# Autodesk Inventor assembly: BeltDrive
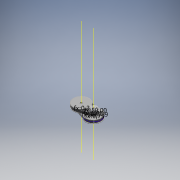
[picture p0: Inventor's stored thumbnail of the model, 180x180]
Saved by Autodesk Inventor 2018.3 (Build 223284000, 284)
## iProperties
Created: 2018-07-29
Part Number: BeltDrive
Material: Generisch
Document SubType Name: Assembly
Designer: JochenAlt
Author: JochenAlt
## Documents named in this file (10)
- D:\Projects\FlowerPot\CAD\Beltdrive\BeltDrive.iam
- D:\Projects\FlowerPot\CAD\Mounting Hub.ipt
- D:\Projects\FlowerPot\CAD\Beltdrive\ZwischenScheibe.ipt
- D:\Projects\FlowerPot\CAD\AST_Bearings_SMR74ZZ.ipt
- D:\Projects\FlowerPot\CAD\Beltdrive\BeltDriveConstruction\Konstruktions-Assistent\Synchrone Riemenscheibe22.ipt
- D:\Projects\FlowerPot\CAD\Beltdrive\Konstruktions-Assistent\Synchrone Riemenscheibe21.ipt
- D:\Projects\FlowerPot\CAD\Beltdrive\Konstruktions-Assistent\Zahnriemen1.ipt
- D:\Projects\FlowerPot\CAD\Beltdrive\BeltDriveConstruction\Konstruktions-Assistent\Zahnriemen2.ipt
- C:\Users\JochenAlt\Documents\Inventor\Content Center Files\R2018\de-DE\DIN 912\DIN 912 - M2,5 x 0,45 x 12 x 10,875.ipt
- C:\Users\JochenAlt\Documents\Inventor\Content Center Files\R2018\de-DE\DIN 912\DIN 912 - M3 x 0,5 x 6 x 4,75.ipt
## Components (17 placed, 8 different names)
1. Mounting Hub:1 — Passend:17, Passend:18, Passend:19, Passend:30
2. BigWheel — Passend:26, Passend:27, Passend:29, Drehung:1, Drehung:2, Fluchtend:2, Fluchtend:3
3. Mounting Hub:2 — Passend:5, Passend:6, Passend:21, Passend:32
4. AST_Bearings_SMR74ZZ:2 — Passend:1, Passend:2
5. AST_Bearings_SMR74ZZ:3 — Passend:3, Passend:4, Passend:16
6. Input — Passend:1, Passend:2, Passend:3, Passend:4, Passend:5, Passend:6, Passend:8, Passend:9, Passend:10, Passend:11, Passend:12, Passend:13, Passend:14, Passend:15, Drehung:1, Passend:31, Passend:32, Fluchtend:3
7. Output — Passend:16, Passend:17, Passend:18, Passend:19, Einfügen:1, Einfügen:2, Einfügen:3, Einfügen:4, Passend:20, Fluchtend:1, Drehung:2, Fluchtend:2
8. Zahnriemen:1 — Passend:20, Passend:23, Passend:24, Passend:29, Fluchtend:1
9. Zahnriemen:2 — Passend:21, Passend:23, Passend:25, Passend:27, Passend:31
10. DIN 912 - ersetzt durch DIN EN ISO 4762 M2,5 x 12:1 — Passend:8, Passend:9
11. DIN 912 - ersetzt durch DIN EN ISO 4762 M2,5 x 12:2 — Passend:10, Passend:11
12. DIN 912 - ersetzt durch DIN EN ISO 4762 M2,5 x 12:3 — Passend:12, Passend:13
13. DIN 912 - ersetzt durch DIN EN ISO 4762 M2,5 x 12:4 — Passend:14, Passend:15
14. DIN 912 - ersetzt durch DIN EN ISO 4762 M3 x 6:1 — Einfügen:1
15. DIN 912 - ersetzt durch DIN EN ISO 4762 M3 x 6:2 — Einfügen:2
16. DIN 912 - ersetzt durch DIN EN ISO 4762 M3 x 6:3 — Einfügen:3
17. DIN 912 - ersetzt durch DIN EN ISO 4762 M3 x 6:4 — Einfügen:4
## Relationships (38: Mate 29, Insert 4, Flush 3, RelateRotation 2)
- Passend:1 [Mate]: AST_Bearings_SMR74ZZ:2 ↔ Input
- Passend:2 [Mate]: AST_Bearings_SMR74ZZ:2 ↔ Input
- Passend:3 [Mate]: AST_Bearings_SMR74ZZ:3 ↔ Input
- Passend:4 [Mate]: AST_Bearings_SMR74ZZ:3 ↔ Input
- Passend:5 [Mate]: Mounting Hub:2 ↔ Input
- Passend:6 [Mate]: Mounting Hub:2 ↔ Input
- Passend:8 [Mate]: Input ↔ DIN 912 - ersetzt durch DIN EN ISO 4762 M2,5 x 12:1
- Passend:9 [Mate]: Input ↔ DIN 912 - ersetzt durch DIN EN ISO 4762 M2,5 x 12:1
- Passend:10 [Mate]: Input ↔ DIN 912 - ersetzt durch DIN EN ISO 4762 M2,5 x 12:2
- Passend:11 [Mate]: Input ↔ DIN 912 - ersetzt durch DIN EN ISO 4762 M2,5 x 12:2
- Passend:12 [Mate]: Input ↔ DIN 912 - ersetzt durch DIN EN ISO 4762 M2,5 x 12:3
- Passend:13 [Mate]: Input ↔ DIN 912 - ersetzt durch DIN EN ISO 4762 M2,5 x 12:3
- Passend:14 [Mate]: Input ↔ DIN 912 - ersetzt durch DIN EN ISO 4762 M2,5 x 12:4
- Passend:15 [Mate]: Input ↔ DIN 912 - ersetzt durch DIN EN ISO 4762 M2,5 x 12:4
- Passend:16 [Mate]: AST_Bearings_SMR74ZZ:3 ↔ Output
- Passend:17 [Mate]: Mounting Hub:1 ↔ Output
- Passend:18 [Mate]: Mounting Hub:1 ↔ Output
- Passend:19 [Mate]: Mounting Hub:1 ↔ Output
- Einfügen:1 [Insert]: Output ↔ DIN 912 - ersetzt durch DIN EN ISO 4762 M3 x 6:1
- Einfügen:2 [Insert]: Output ↔ DIN 912 - ersetzt durch DIN EN ISO 4762 M3 x 6:2
- Einfügen:3 [Insert]: Output ↔ DIN 912 - ersetzt durch DIN EN ISO 4762 M3 x 6:3
- Einfügen:4 [Insert]: Output ↔ DIN 912 - ersetzt durch DIN EN ISO 4762 M3 x 6:4
- Passend:20 [Mate]: Output ↔ Zahnriemen:1
- Passend:21 [Mate]: Mounting Hub:2 ↔ Zahnriemen:2
- Passend:23 [Mate]: Zahnriemen:1 ↔ Zahnriemen:2
- Passend:24 [Mate]: Zahnriemen:1
- Passend:25 [Mate]: Zahnriemen:2
- Passend:26 [Mate]: BigWheel
- Passend:27 [Mate] (31.8 mm): BigWheel ↔ Zahnriemen:2
- Passend:29 [Mate] (0.75 mm): BigWheel ↔ Zahnriemen:1
- Fluchtend:1 [Flush] (-0.75 mm): Output ↔ Zahnriemen:1
- Passend:30 [Mate]: Mounting Hub:1
- Drehung:1 [RelateRotation] (0.48 ul): BigWheel ↔ Input
- Drehung:2 [RelateRotation] (0.48 ul): BigWheel ↔ Output
- Passend:31 [Mate] (0.75 mm): Input ↔ Zahnriemen:2
- Passend:32 [Mate]: Mounting Hub:2 ↔ Input
- Fluchtend:2 [Flush]: BigWheel ↔ Output
- Fluchtend:3 [Flush]: BigWheel ↔ Input
